# Autodesk Inventor assembly: ModuloMeson
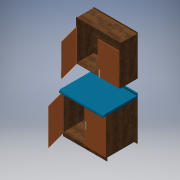
[picture p0: Inventor's stored thumbnail of the model, 180x180]
Saved by Autodesk Inventor 2016 (Build 200138000, 138)
## iProperties
Created: 2015-11-25
Part Number: ModuloMeson
Document SubType Name: Assembly
Designer: Daniela
Author: Daniela
## Documents named in this file (5)
- D:\Documents\Carrera\11.Semeste_II_2015\Computacion_grafica\Proyecto\COCINA_FINAL\Cocina\ModuloMeson.iam
- D:\Documents\Carrera\11.Semeste_II_2015\Computacion_grafica\Proyecto\COCINA_FINAL\Cocina\esqueleto.ipt
- D:\Documents\Carrera\11.Semeste_II_2015\Computacion_grafica\Proyecto\COCINA_FINAL\Cocina\pared.ipt
- D:\Documents\Carrera\11.Semeste_II_2015\Computacion_grafica\Proyecto\COCINA_FINAL\Cocina\puertas.iam
- D:\Documents\Carrera\11.Semeste_II_2015\Computacion_grafica\Proyecto\COCINA_FINAL\Cocina\meson.ipt
## Components (5 placed, 4 different names)
1. esqueleto:1 — Mate:3, Mate:4, Coincidencia:5, Coincidencia:6, Coincidencia:7, Nivelación:1, Mate:9, Flush:2
2. pared:1 — Coincidencia:5, Coincidencia:6, Coincidencia:8, Flush:3
3. pared:2 — Mate:3, Mate:4
4. puertas:1 [sub-assembly] — Coincidencia:7, Nivelación:1, Coincidencia:8
5. meson:1 — Mate:9, Flush:2, Flush:3
## Relationships (10: Mate 7, Flush 3)
- Mate:3: esqueleto:1 ↔ pared:2
- Mate:4: esqueleto:1 ↔ pared:2
- Coincidencia:5 [Mate]: esqueleto:1 ↔ pared:1
- Coincidencia:6 [Mate]: esqueleto:1 ↔ pared:1
- Coincidencia:7 [Mate]: esqueleto:1 ↔ puertas:1
- Nivelación:1 [Flush] (70 mm): esqueleto:1 ↔ puertas:1
- Coincidencia:8 [Mate] (10 mm): pared:1 ↔ puertas:1
- Mate:9: esqueleto:1 ↔ meson:1
- Flush:2: esqueleto:1 ↔ meson:1
- Flush:3: pared:1 ↔ meson:1
